# Autodesk Inventor assembly: Robot
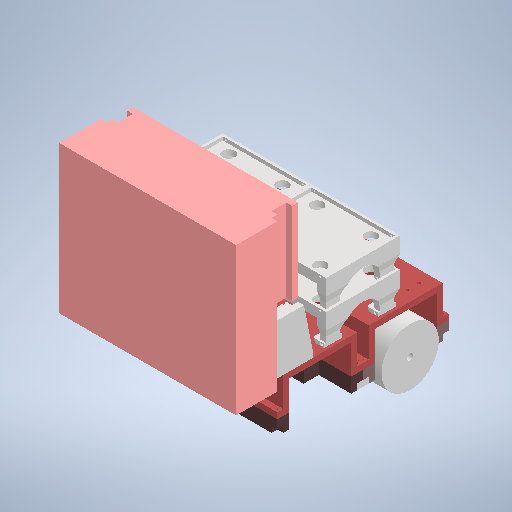
[picture p0: Inventor's stored thumbnail of the model, 512x512]
Saved by Autodesk Inventor 2025.3 (Build 293356000, 356)
## iProperties
Created: 2025-04-27
Part Number: Robot
Document SubType Name: Assembly
Designer: SEON
Author: SEON
## Documents named in this file (13)
- C:\Users\SEON\Documents\Inventor\LastCapstone\Robot.iam
- C:\Users\SEON\Documents\Inventor\LastCapstone\DummyModule.ipt
- C:\Users\SEON\Documents\Inventor\LastCapstone\RobotBase.ipt
- C:\Users\SEON\Documents\Inventor\LastCapstone\DummyWheel.ipt
- C:\Users\SEON\Documents\Inventor\LastCapstone\WheelCorver.ipt
- C:\Users\SEON\Documents\Inventor\LastCapstone\partContainer.ipt
- C:\Users\SEON\Documents\Inventor\LastCapstone\partContainerConnector.ipt
- C:\Users\SEON\Documents\Inventor\LastCapstone\RobotBaseConnector.ipt
- C:\Users\SEON\Documents\Inventor\LastCapstone\RobotBaseConnector1x2.ipt
- C:\Users\SEON\Documents\Inventor\LastCapstone\NewModuleConnectorLeft.ipt
- C:\Users\SEON\Documents\Inventor\LastCapstone\NewModuleConnectorRight.ipt
- C:\Users\SEON\Documents\Inventor\LastCapstone\motor.ipt
- C:\Users\SEON\Documents\Inventor\LastCapstone\MotorCover.ipt
## Components (31 placed, 12 different names)
1. RobotBase:1 — 메이트:1, 메이트:4, 메이트:5, 메이트:6, 메이트:9, 플러쉬:4, 메이트:11, 메이트:12, 플러쉬:5, 플러쉬:6, 메이트:13, 플러쉬:8, 플러쉬:17, 메이트:29, 플러쉬:18, 메이트:67, 메이트:69, 메이트:71, 메이트:79
2. DummyModule:1 — 메이트:6, 메이트:84, 메이트:85
3. DummyWheel:1 — 각도:1, 메이트:88
4. WheelCorver:1 — 메이트:9, 플러쉬:4, 플러쉬:10, 플러쉬:11, 메이트:17, 메이트:21, 플러쉬:14, 메이트:30, 메이트:34, 메이트:41, 메이트:81, 플러쉬:23, 메이트:82
5. WheelCorver:2 — 메이트:11, 플러쉬:11, 메이트:17, 메이트:26, 메이트:33, 메이트:37, 메이트:38
6. RobotBase:2 — 메이트:13, 메이트:15, 플러쉬:7, 플러쉬:8, 플러쉬:10, 메이트:72, 메이트:74, 메이트:75, 메이트:80
7. RobotBase:3 — 메이트:14, 메이트:15, 플러쉬:7, 플러쉬:9, 메이트:73, 메이트:77, 플러쉬:26, 메이트:89, 메이트:90, 메이트:91
8. RobotBase:4 — 메이트:12, 플러쉬:5, 플러쉬:6, 메이트:14, 플러쉬:9, 메이트:28, 플러쉬:15, 플러쉬:16, 메이트:66, 메이트:68, 메이트:70, 메이트:76, 메이트:78
9. partContainer:1 — 메이트:20, 플러쉬:12, 플러쉬:13, 메이트:21, 플러쉬:14, 메이트:25, 메이트:27, 메이트:31, 메이트:32, 메이트:35, 메이트:36, 메이트:39, 메이트:40, 메이트:42, 메이트:44, 메이트:45
10. partContainer:2 — 메이트:20, 플러쉬:12, 플러쉬:13, 메이트:43, 메이트:46, 메이트:47, 메이트:48, 메이트:49, 메이트:51, 메이트:52, 메이트:54, 메이트:55, 플러쉬:19, 메이트:56, 플러쉬:20, 메이트:57
11. partContainer:4 — 메이트:43, 메이트:46, 메이트:47
12. partContainerConnector:1 — 메이트:25, 메이트:26, 메이트:27, 메이트:33
13. WheelCorver:3 — 메이트:28, 플러쉬:15, 플러쉬:16, 메이트:50
14. WheelCorver:4 — 플러쉬:17, 메이트:29, 플러쉬:18, 메이트:53, 메이트:83, 플러쉬:24, 플러쉬:25
15. partContainerConnector:2 — 메이트:30, 메이트:31, 메이트:32, 메이트:34
16. partContainerConnector:3 — 메이트:35, 메이트:36, 메이트:37, 메이트:38
17. partContainerConnector:4 — 메이트:39, 메이트:40, 메이트:41
18. partContainer:5 — 메이트:42, 메이트:44, 메이트:45
19. partContainerConnector:5 — 메이트:48, 메이트:49, 메이트:50
20. partContainerConnector:6 — 메이트:51, 메이트:52, 메이트:53
21. partContainerConnector:7 — 메이트:56, 플러쉬:20, 메이트:57
22. partContainerConnector:8 — 메이트:54, 메이트:55, 플러쉬:19
23. RobotBaseConnector:1 — 메이트:66, 메이트:67, 메이트:68
24. RobotBaseConnector1x2:1 — 메이트:72, 메이트:73, 메이트:74
25. RobotBaseConnector1x2:2 — 메이트:69, 메이트:70, 메이트:71
26. RobotBaseConnector1x2:3 — 메이트:76, 메이트:77, 메이트:78
27. RobotBaseConnector1x2:4 — 메이트:75, 메이트:79, 메이트:80
28. NewModuleConnectorLeft:1 — 메이트:81, 플러쉬:23, 메이트:82, 메이트:85
29. NewModuleConnectorRight:1 — 메이트:83, 플러쉬:24, 플러쉬:25, 메이트:84
30. motor:1 — 메이트:86, 메이트:87, 메이트:88
31. MotorCover:1 — 메이트:86, 메이트:87, 플러쉬:26, 메이트:89, 메이트:90, 메이트:91
## Relationships (94: Mate 72, Flush 21, Angle 1)
- 메이트:1 [Mate]: RobotBase:1
- 메이트:4 [Mate]: RobotBase:1
- 메이트:5 [Mate]: RobotBase:1
- 메이트:6 [Mate]: RobotBase:1 ↔ DummyModule:1
- 각도:1 [Angle] (0 deg): DummyWheel:1
- 메이트:9 [Mate]: RobotBase:1 ↔ WheelCorver:1
- 플러쉬:4 [Flush]: RobotBase:1 ↔ WheelCorver:1
- 메이트:11 [Mate]: RobotBase:1 ↔ WheelCorver:2
- 메이트:12 [Mate]: RobotBase:1 ↔ RobotBase:4
- 플러쉬:5 [Flush]: RobotBase:1 ↔ RobotBase:4
- 플러쉬:6 [Flush]: RobotBase:1 ↔ RobotBase:4
- 메이트:13 [Mate]: RobotBase:1 ↔ RobotBase:2
- 메이트:14 [Mate]: RobotBase:3 ↔ RobotBase:4
- 메이트:15 [Mate]: RobotBase:2 ↔ RobotBase:3
- 플러쉬:7 [Flush]: RobotBase:2 ↔ RobotBase:3
- 플러쉬:8 [Flush]: RobotBase:1 ↔ RobotBase:2
- 플러쉬:9 [Flush]: RobotBase:3 ↔ RobotBase:4
- 플러쉬:10 [Flush]: WheelCorver:1 ↔ RobotBase:2
- 플러쉬:11 [Flush]: WheelCorver:1 ↔ WheelCorver:2
- 메이트:17 [Mate]: WheelCorver:1 ↔ WheelCorver:2
- 메이트:20 [Mate]: partContainer:1 ↔ partContainer:2
- 플러쉬:12 [Flush]: partContainer:1 ↔ partContainer:2
- 플러쉬:13 [Flush]: partContainer:1 ↔ partContainer:2
- 메이트:21 [Mate]: WheelCorver:1 ↔ partContainer:1
- 플러쉬:14 [Flush]: WheelCorver:1 ↔ partContainer:1
- 메이트:25 [Mate]: partContainer:1 ↔ partContainerConnector:1
- 메이트:26 [Mate]: WheelCorver:2 ↔ partContainerConnector:1
- 메이트:27 [Mate]: partContainer:1 ↔ partContainerConnector:1
- 메이트:28 [Mate]: RobotBase:4 ↔ WheelCorver:3
- 플러쉬:15 [Flush]: RobotBase:4 ↔ WheelCorver:3
- 플러쉬:16 [Flush]: RobotBase:4 ↔ WheelCorver:3
- 플러쉬:17 [Flush]: RobotBase:1 ↔ WheelCorver:4
- 메이트:29 [Mate]: RobotBase:1 ↔ WheelCorver:4
- 플러쉬:18 [Flush]: RobotBase:1 ↔ WheelCorver:4
- 메이트:30 [Mate]: WheelCorver:1 ↔ partContainerConnector:2
- 메이트:31 [Mate]: partContainer:1 ↔ partContainerConnector:2
- 메이트:32 [Mate]: partContainer:1 ↔ partContainerConnector:2
- 메이트:33 [Mate]: WheelCorver:2 ↔ partContainerConnector:1
- 메이트:34 [Mate]: WheelCorver:1 ↔ partContainerConnector:2
- 메이트:35 [Mate]: partContainer:1 ↔ partContainerConnector:3
- 메이트:36 [Mate]: partContainer:1 ↔ partContainerConnector:3
- 메이트:37 [Mate]: WheelCorver:2 ↔ partContainerConnector:3
- 메이트:38 [Mate]: WheelCorver:2 ↔ partContainerConnector:3
- 메이트:39 [Mate]: partContainer:1 ↔ partContainerConnector:4
- 메이트:40 [Mate]: partContainer:1 ↔ partContainerConnector:4
- 메이트:41 [Mate]: WheelCorver:1 ↔ partContainerConnector:4
- 메이트:42 [Mate]: partContainer:1 ↔ partContainer:5
- 메이트:43 [Mate]: partContainer:2 ↔ partContainer:4
- 메이트:44 [Mate] (0.5 mm): partContainer:1 ↔ partContainer:5
- 메이트:45 [Mate] (0.5 mm): partContainer:1 ↔ partContainer:5
- 메이트:46 [Mate] (0.5 mm): partContainer:2 ↔ partContainer:4
- 메이트:47 [Mate] (0.5 mm): partContainer:2 ↔ partContainer:4
- 메이트:48 [Mate]: partContainer:2 ↔ partContainerConnector:5
- 메이트:49 [Mate]: partContainer:2 ↔ partContainerConnector:5
- 메이트:50 [Mate]: WheelCorver:3 ↔ partContainerConnector:5
- 메이트:51 [Mate]: partContainer:2 ↔ partContainerConnector:6
- 메이트:52 [Mate]: partContainer:2 ↔ partContainerConnector:6
- 메이트:53 [Mate]: WheelCorver:4 ↔ partContainerConnector:6
- 메이트:54 [Mate]: partContainer:2 ↔ partContainerConnector:8
- 메이트:55 [Mate]: partContainer:2 ↔ partContainerConnector:8
- 플러쉬:19 [Flush]: partContainer:2 ↔ partContainerConnector:8
- 메이트:56 [Mate]: partContainer:2 ↔ partContainerConnector:7
- 플러쉬:20 [Flush]: partContainer:2 ↔ partContainerConnector:7
- 메이트:57 [Mate]: partContainer:2 ↔ partContainerConnector:7
- 메이트:66 [Mate]: RobotBase:4 ↔ RobotBaseConnector:1
- 메이트:67 [Mate]: RobotBase:1 ↔ RobotBaseConnector:1
- 메이트:68 [Mate]: RobotBase:4 ↔ RobotBaseConnector:1
- 메이트:69 [Mate]: RobotBase:1 ↔ RobotBaseConnector1x2:2
- 메이트:70 [Mate]: RobotBase:4 ↔ RobotBaseConnector1x2:2
- 메이트:71 [Mate]: RobotBase:1 ↔ RobotBaseConnector1x2:2
- 메이트:72 [Mate]: RobotBase:2 ↔ RobotBaseConnector1x2:1
- 메이트:73 [Mate]: RobotBase:3 ↔ RobotBaseConnector1x2:1
- 메이트:74 [Mate]: RobotBase:2 ↔ RobotBaseConnector1x2:1
- 메이트:75 [Mate]: RobotBase:2 ↔ RobotBaseConnector1x2:4
- 메이트:76 [Mate]: RobotBase:4 ↔ RobotBaseConnector1x2:3
- 메이트:77 [Mate]: RobotBase:3 ↔ RobotBaseConnector1x2:3
- 메이트:78 [Mate]: RobotBase:4 ↔ RobotBaseConnector1x2:3
- 메이트:79 [Mate]: RobotBase:1 ↔ RobotBaseConnector1x2:4
- 메이트:80 [Mate]: RobotBase:2 ↔ RobotBaseConnector1x2:4
- 메이트:81 [Mate]: WheelCorver:1 ↔ NewModuleConnectorLeft:1
- 플러쉬:23 [Flush]: WheelCorver:1 ↔ NewModuleConnectorLeft:1
- 메이트:82 [Mate]: WheelCorver:1 ↔ NewModuleConnectorLeft:1
- 메이트:83 [Mate]: WheelCorver:4 ↔ NewModuleConnectorRight:1
- 플러쉬:24 [Flush]: WheelCorver:4 ↔ NewModuleConnectorRight:1
- 플러쉬:25 [Flush]: WheelCorver:4 ↔ NewModuleConnectorRight:1
- 메이트:84 [Mate]: DummyModule:1 ↔ NewModuleConnectorRight:1
- 메이트:85 [Mate]: DummyModule:1 ↔ NewModuleConnectorLeft:1
- 메이트:86 [Mate]: motor:1 ↔ MotorCover:1
- 메이트:87 [Mate]: motor:1 ↔ MotorCover:1
- 플러쉬:26 [Flush]: RobotBase:3 ↔ MotorCover:1
- 메이트:88 [Mate]: DummyWheel:1 ↔ motor:1
- 메이트:89 [Mate]: RobotBase:3 ↔ MotorCover:1
- 메이트:90 [Mate]: RobotBase:3 ↔ MotorCover:1
- 메이트:91 [Mate]: RobotBase:3 ↔ MotorCover:1
